# Autodesk Inventor assembly: BevelTo20TSpureGear
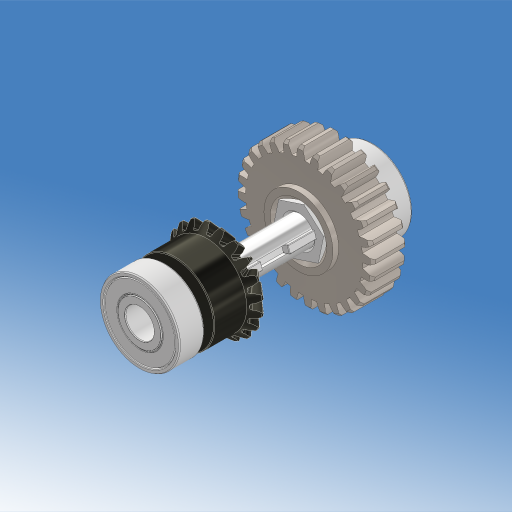
[picture p0: Inventor's stored thumbnail of the model, 512x512]
Saved by Autodesk Inventor 2024 (Build 280153000, 153)
## iProperties
Created: 2024-04-23
Part Number: BevelTo20TSpureGear
Document SubType Name: Assembly
Designer: seene
Author: seene
## Documents named in this file (7)
- C:\Users\seene\OneDrive\SBRT\Robocup Rescue\Drive\v1\BevelTo20TSpureGear.iam
- C:\Users\seene\OneDrive\SBRT\Robocup Rescue\Drive\v1\1439K211_1045 Carbon Steel Keyed Rotary Shaft.ipt
- C:\Users\seene\OneDrive\SBRT\Robocup Rescue\Drive\v1\am-3776 Miter Gear 1.25, 20T, 8mm, 2mm Key Bore.ipt
- C:\Users\seene\OneDrive\SBRT\Robocup Rescue\Drive\v1\am-0588_short 8mm 500 Hex Adapter Shaft 500 long.ipt
- C:\Users\seene\OneDrive\SBRT\Robocup Rescue\Drive\v1\Gears\am-5133 28T 20DP 500hex 375 FW.ipt
- C:\Users\seene\OneDrive\SBRT\Robocup Rescue\Drive\v1\98870A702_Machine Key.ipt
- C:\Users\seene\OneDrive\SBRT\Robocup Rescue\Drive\v1\2349K744_Permanently Lubricated Ball Bearing.ipt
## Components (8 placed, 6 different names)
1. 1439K211_1045 Carbon Steel Keyed Rotary Shaft:1 — Mate:1, Flush:1, Mate:2, Flush:3, Mate:9, Mate:10, Flush:7
2. am-3776 Miter Gear 1.25, 20T, 8mm, 2mm Key Bore:1 — Mate:1, Flush:1, Mate:5, Mate:6, Mate:13
3. am-0588_short 8mm 500 Hex Adapter Shaft 500 long:1 — Mate:2, Flush:3, Mate:3, Mate:4, Flush:4, Mate:7, Mate:8, Flush:6
4. am-5133 28T 20DP 500hex 375 FW:1 — Mate:3, Mate:4, Flush:4, Mate:12
5. 98870A702_Machine Key:1 — Mate:5, Mate:6
6. 98870A702_Machine Key:2 — Mate:7, Mate:8, Flush:6
7. 2349K744_Permanently Lubricated Ball Bearing:1 — Mate:9, Mate:11, Mate:13
8. 2349K744_Permanently Lubricated Ball Bearing:2 — Mate:10, Flush:7, Mate:11, Mate:12
## Relationships (18: Mate 13, Flush 5)
- Mate:1: 1439K211_1045 Carbon Steel Keyed Rotary Shaft:1 ↔ am-3776 Miter Gear 1.25, 20T, 8mm, 2mm Key Bore:1
- Flush:1: 1439K211_1045 Carbon Steel Keyed Rotary Shaft:1 ↔ am-3776 Miter Gear 1.25, 20T, 8mm, 2mm Key Bore:1
- Mate:2: 1439K211_1045 Carbon Steel Keyed Rotary Shaft:1 ↔ am-0588_short 8mm 500 Hex Adapter Shaft 500 long:1
- Flush:3: 1439K211_1045 Carbon Steel Keyed Rotary Shaft:1 ↔ am-0588_short 8mm 500 Hex Adapter Shaft 500 long:1
- Mate:3: am-0588_short 8mm 500 Hex Adapter Shaft 500 long:1 ↔ am-5133 28T 20DP 500hex 375 FW:1
- Mate:4: am-0588_short 8mm 500 Hex Adapter Shaft 500 long:1 ↔ am-5133 28T 20DP 500hex 375 FW:1
- Flush:4: am-0588_short 8mm 500 Hex Adapter Shaft 500 long:1 ↔ am-5133 28T 20DP 500hex 375 FW:1
- Mate:5: am-3776 Miter Gear 1.25, 20T, 8mm, 2mm Key Bore:1 ↔ 98870A702_Machine Key:1
- Mate:6: am-3776 Miter Gear 1.25, 20T, 8mm, 2mm Key Bore:1 ↔ 98870A702_Machine Key:1
- Mate:7: am-0588_short 8mm 500 Hex Adapter Shaft 500 long:1 ↔ 98870A702_Machine Key:2
- Mate:8: am-0588_short 8mm 500 Hex Adapter Shaft 500 long:1 ↔ 98870A702_Machine Key:2
- Flush:6: am-0588_short 8mm 500 Hex Adapter Shaft 500 long:1 ↔ 98870A702_Machine Key:2
- Mate:9: 1439K211_1045 Carbon Steel Keyed Rotary Shaft:1 ↔ 2349K744_Permanently Lubricated Ball Bearing:1
- Mate:10: 1439K211_1045 Carbon Steel Keyed Rotary Shaft:1 ↔ 2349K744_Permanently Lubricated Ball Bearing:2
- Flush:7: 1439K211_1045 Carbon Steel Keyed Rotary Shaft:1 ↔ 2349K744_Permanently Lubricated Ball Bearing:2
- Mate:11 (50.8 mm): 2349K744_Permanently Lubricated Ball Bearing:1 ↔ 2349K744_Permanently Lubricated Ball Bearing:2
- Mate:12 (0.7937 mm): am-5133 28T 20DP 500hex 375 FW:1 ↔ 2349K744_Permanently Lubricated Ball Bearing:2
- Mate:13 (13.8268 mm): am-3776 Miter Gear 1.25, 20T, 8mm, 2mm Key Bore:1 ↔ 2349K744_Permanently Lubricated Ball Bearing:1
